# Autodesk Inventor assembly: main_frame_assem
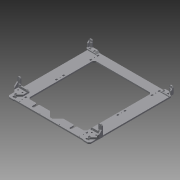
[picture p0: Inventor's stored thumbnail of the model, 180x180]
Saved by Autodesk Inventor 2015 (Build 190159000, 159)
## iProperties
Created: 2015-06-01
Part Number: main_frame_assem
Document SubType Name: Assembly
Designer: X
Author: X
## Documents named in this file (6)
- G:\3d printer\Prusa_i3\CAD\main_frame_assem.iam
- G:\3d printer\Prusa_i3\CAD\frame\main_frame.ipt
- G:\3d printer\Prusa_i3\CAD\3d_printer_part\z-axis-top.ipt
- G:\3d printer\Prusa_i3\CAD\3d_printer_part\z-axis-bottom.ipt
- G:\3d printer\Prusa_i3\CAD\3d_printer_part\z-axis-top_MIR.ipt
- G:\3d printer\Prusa_i3\CAD\3d_printer_part\z-axis-bottom_MIR.ipt
## Components (5 placed, 5 different names)
1. main_frame:1 — Mate:1, Cylindrical:1, Cylindrical:2, Mate:2, Cylindrical:3, Cylindrical:4, Mate:3, Mate:4
2. z-axis-top:1 — Mate:1, Cylindrical:1, Cylindrical:2
3. z-axis-bottom:1 — Mate:2, Cylindrical:3, Cylindrical:4
4. z-axis-top_MIR:1
5. z-axis-bottom_MIR:1
## Relationships (9: Mate 4, CylindricalJoint 4, Flush 1)
- Mate:1: main_frame:1 ↔ z-axis-top:1
- Cylindrical:1: main_frame:1 ↔ z-axis-top:1
- Cylindrical:2: main_frame:1 ↔ z-axis-top:1
- Mate:2: main_frame:1 ↔ z-axis-bottom:1
- Cylindrical:3: main_frame:1 ↔ z-axis-bottom:1
- Cylindrical:4: main_frame:1 ↔ z-axis-bottom:1
- Mate:3: main_frame:1
- Mate:4: main_frame:1
- Flush:1 (185 mm)
